# Autodesk Inventor assembly: Whack01-Assembly
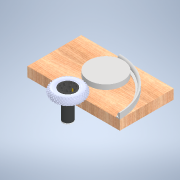
[picture p0: Inventor's stored thumbnail of the model, 180x180]
Saved by Autodesk Inventor 2022 (Build 260153000, 153)
## iProperties
Created: 2021-04-23
Part Number: Whack01-Assembly
Document SubType Name: Assembly
Designer: robst
Author: robst
## Documents named in this file (9)
- C:\git\CAD-Development\robSteele\2021 Frisbee Robot\Whack01-Assembly.iam
- C:\git\CAD-Development\robSteele\2021 Frisbee Robot\am-4244 1IN Bent Bearing Side Mount Gusset.ipt
- C:\git\CAD-Development\robSteele\2021 Frisbee Robot\am-0255 2.5inch CIM Motor.ipt
- C:\git\CAD-Development\robSteele\2021 Frisbee Robot\am-4119 8mm Key Hub.ipt
- C:\git\CAD-Development\robSteele\2021 Frisbee Robot\PneumaticWheel_am-0970.iam
- C:\git\CAD-Development\robSteele\2021 Frisbee Robot\Whack01-BaseForFrisbeeShooter.ipt
- C:\git\CAD-Development\robSteele\2021 Frisbee Robot\Whack01-RunnerForFrisbeeShooter.ipt
- C:\git\CAD-Development\robSteele\2021 Frisbee Robot\frisbee_9_000.ipt
- C:\git\CAD-Development\robSteele\2021 Frisbee Robot\simulatedWheel.ipt
## Components (8 placed, 8 different names)
1. am-4244 1IN Bent Bearing Side Mount Gusset:1 — Insert:1, Insert:2, Insert:3, Mate:1, Flush:1, Flush:2
2. am-0255 2.5inch CIM Motor:1 — Insert:1, Insert:2, Insert:3, Insert:4
3. am-4119 8mm Key Hub:1 — Insert:4, Insert:5
4. PneumaticWheel_am-0970:1 [sub-assembly] — Insert:5, Insert:6
5. Whack01-BaseForFrisbeeShooter:1 — Mate:1, Flush:1, Flush:2, Mate:2, Flush:3
6. Whack01-RunnerForFrisbeeShooter:1 — Mate:2, Flush:3
7. frisbee_9_000:1 — Tangent:1
8. simulatedWheel:1 — Insert:6, Tangent:1
## Relationships (12: Insert 6, Flush 3, Mate 2, Tangent 1)
- Insert:1: am-4244 1IN Bent Bearing Side Mount Gusset:1 ↔ am-0255 2.5inch CIM Motor:1
- Insert:2: am-4244 1IN Bent Bearing Side Mount Gusset:1 ↔ am-0255 2.5inch CIM Motor:1
- Insert:3: am-4244 1IN Bent Bearing Side Mount Gusset:1 ↔ am-0255 2.5inch CIM Motor:1
- Insert:4: am-0255 2.5inch CIM Motor:1 ↔ am-4119 8mm Key Hub:1
- Insert:5: am-4119 8mm Key Hub:1 ↔ PneumaticWheel_am-0970:1
- Mate:1: am-4244 1IN Bent Bearing Side Mount Gusset:1 ↔ Whack01-BaseForFrisbeeShooter:1
- Flush:1 (-22.225 mm): am-4244 1IN Bent Bearing Side Mount Gusset:1 ↔ Whack01-BaseForFrisbeeShooter:1
- Flush:2 (260.35 mm): am-4244 1IN Bent Bearing Side Mount Gusset:1 ↔ Whack01-BaseForFrisbeeShooter:1
- Mate:2: Whack01-BaseForFrisbeeShooter:1 ↔ Whack01-RunnerForFrisbeeShooter:1
- Insert:6: PneumaticWheel_am-0970:1 ↔ simulatedWheel:1
- Tangent:1: frisbee_9_000:1 ↔ simulatedWheel:1
- Flush:3: Whack01-BaseForFrisbeeShooter:1 ↔ Whack01-RunnerForFrisbeeShooter:1
